# Autodesk Inventor assembly: HP2 Raceparts
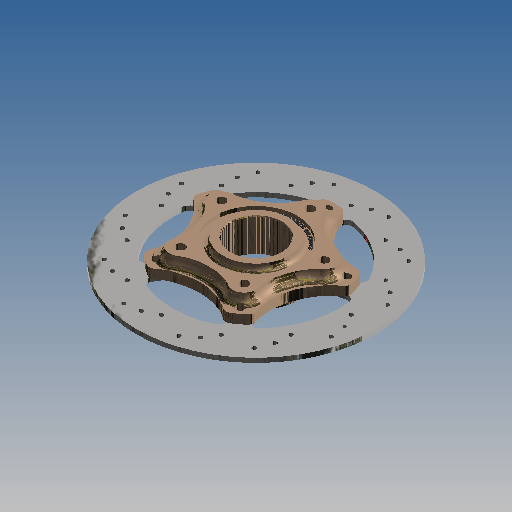
[picture p0: Inventor's stored thumbnail of the model, 512x512]
Saved by Autodesk Inventor 2017.2 (Build 212233000, 233)
## iProperties
Created: 2017-01-15
Part Number: HP2 Raceparts
Material: Generisch
Document SubType Name: Assembly
Designer: Catweazle
Author: Catweazle
## Documents named in this file (3)
- K:\BMW HP2 Raceparts\HP2 Raceparts.iam
- K:\BMW HP2 Raceparts\HP2 Raceparts 002.ipt
- K:\BMW HP2 Raceparts\HP2 Raceparts 001.ipt
## Components (2 placed, 2 different names)
1. HP2 Raceparts 002:1 — Passend:1, Passend:2, Passend:3
2. HP2 Raceparts 001:1 — Passend:1, Passend:2, Passend:3
## Relationships (3: Mate 3)
- Passend:1 [Mate]: HP2 Raceparts 002:1 ↔ HP2 Raceparts 001:1
- Passend:2 [Mate]: HP2 Raceparts 002:1 ↔ HP2 Raceparts 001:1
- Passend:3 [Mate]: HP2 Raceparts 002:1 ↔ HP2 Raceparts 001:1
